# Autodesk Inventor assembly: Baugruppe1
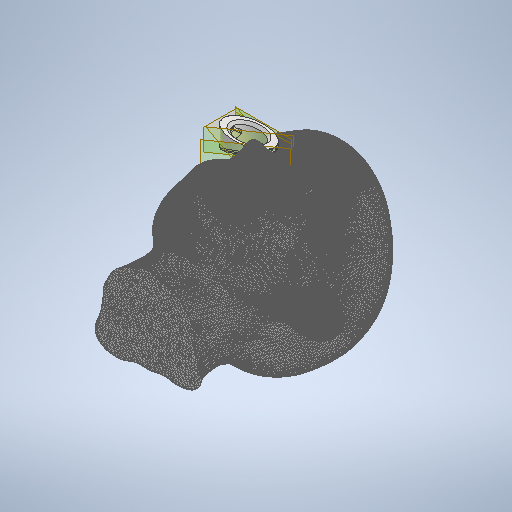
[picture p0: Inventor's stored thumbnail of the model, 512x512]
Saved by Autodesk Inventor 2025.1 (Build 291241000, 241)
## iProperties
Created: 2025-02-01
Part Number: Baugruppe1
Document SubType Name: Assembly
Designer: joebe
Author: joebe
## Documents named in this file (6)
- C:\Users\joebe\OneDrive\Documents\Projekte\Macrolampe\CAD\Baugruppen\Baugruppe1.iam
- C:\Users\joebe\OneDrive\Documents\Projekte\Macrolampe\CAD\Einzelteile\Gesichtshalter.ipt
- C:\Users\joebe\OneDrive\Documents\Projekte\Macrolampe\CAD\Einzelteile\iiihead.ipt
- C:\Users\joebe\OneDrive\Documents\Projekte\Macrolampe\CAD\Baugruppen\Macrolight.iam
- C:\Users\joebe\OneDrive\Documents\Projekte\Macrolampe\CAD\Einzelteile\RundesLicht.ipt
- C:\Users\joebe\OneDrive\Documents\Projekte\Macrolampe\CAD\Einzelteile\iiihead\iiihead\iiihead.ipt
## Components (6 placed, 4 different names)
1. Gesichtshalter:1 — Passend:1, Winkel:1
2. iiihead:1
3. Macrolight:3 [sub-assembly] — Passend:1, Winkel:1
4. RundesLicht:1 — Fluchtend:1, Fluchtend:2
5. iiihead:2
6. iiihead:3
## Relationships (4: Flush 2, Mate 1, Angle 1)
- Passend:1 [Mate] (100 mm): Gesichtshalter:1 ↔ Macrolight:3
- Winkel:1 [Angle] (0 deg): Gesichtshalter:1 ↔ Macrolight:3
- Fluchtend:1 [Flush]: RundesLicht:1
- Fluchtend:2 [Flush]: RundesLicht:1
